# Autodesk Inventor assembly: IG-42GM+Encoder(49ratio)
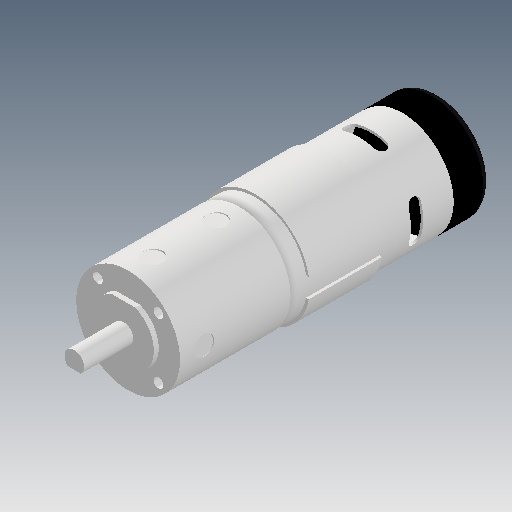
[picture p0: Inventor's stored thumbnail of the model, 512x512]
Saved by Autodesk Inventor 2020 (Build 240168000, 168)
## iProperties
Created: 2020-08-28
Part Number: IG-42GM+Encoder(49ratio)
Document SubType Name: Assembly
Designer: 이호석
Mass: 591 g
Surface Area: 419.64 cm^2
Volume: 100.801 cm^3
Density: 5.86304 g/cm^3
Author: 이호석
## Documents named in this file (6)
- C:\Inventor\Embedded_contest\ig42gm\IG-42GM+Encoder(49ratio).iam
- C:\Inventor\Embedded_contest\ig42gm\motor.ipt
- C:\Inventor\Embedded_contest\ig42gm\encoder.ipt
- C:\Inventor\Embedded_contest\ig42gm\shaft.ipt
- C:\Inventor\Embedded_contest\ig42gm\gear(49ratio).ipt
- C:\Inventor\Embedded_contest\ig42gm\case.ipt
## Components (5 placed, 5 different names)
1. motor:1 — 메이트:1, 삽입:1, 플러쉬:1, 삽입:3, 플러쉬:2
2. encoder:1 — 메이트:1, 삽입:1
3. case:1 — 플러쉬:1, 삽입:5
4. gear(49ratio):1 — 삽입:3, 플러쉬:2, 삽입:4, 삽입:5
5. shaft:1 — 삽입:4
## Relationships (7: Insert 4, Flush 2, Mate 1)
- 메이트:1 [Mate]: motor:1 ↔ encoder:1
- 삽입:1 [Insert]: motor:1 ↔ encoder:1
- 플러쉬:1 [Flush]: motor:1 ↔ case:1
- 삽입:3 [Insert]: motor:1 ↔ gear(49ratio):1
- 플러쉬:2 [Flush] (-15.5 mm): motor:1 ↔ gear(49ratio):1
- 삽입:4 [Insert]: gear(49ratio):1 ↔ shaft:1
- 삽입:5 [Insert] (6 mm): case:1 ↔ gear(49ratio):1
